# Autodesk Inventor assembly: 72 to 12 Single Stage Gearbox
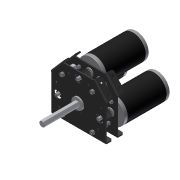
[picture p0: Inventor's stored thumbnail of the model, 180x180]
Saved by Autodesk Inventor 2013 (Build 170138000, 138)
## iProperties
Created: 2013-01-07
Part Number: 72 to 12 Single Stage Gearbox
Document SubType Name: Assembly
Designer: Nemo
Author: Nemo
## Documents named in this file (10)
- H:\Nemo\Documents\Robotics\VexPro\Gearbox - Single Reduction\72 to 12 Single Stage Gearbox.iam
- H:\Nemo\Documents\Robotics\VexPro\Gearbox - Single Reduction\72 single stage gearbox plate.ipt
- H:\Nemo\Documents\Robotics\VexPro\Fasteners\Hex Standoff 14-20 x1000.ipt
- H:\Nemo\Documents\Robotics\COTS Parts\Fasteners\14-20 SHCS x500.ipt
- H:\Nemo\Documents\Robotics\VexPro\Gearbox - Single Reduction\Single stage gearbox output shaft.ipt
- H:\Nemo\Documents\Robotics\VexPro\Bearings\Flanged Bearing - 0.5in Hex ID x 1.125in OD.ipt
- H:\Nemo\Documents\Robotics\VexPro\Bearings\Flanged Bearing - 0.5in Round ID x 1.125in OD.ipt
- H:\Nemo\Documents\Robotics\VexPro\Gears\Gear 20dp 500hex 72T Vex.ipt
- H:\Nemo\Documents\Robotics\VexPro\Gearbox - Single Reduction\500 Hex Coupler.ipt
- H:\Nemo\Documents\Robotics\VexPro\Gearbox - Single Reduction\CIM for Single Stage Vex Box.iam
## Components (22 placed, 9 different names)
1. 72 single stage gearbox plate:1 — Mate:1, Mate:2, Insert:1, Insert:2, Insert:3, Insert:4, Mate:3, Insert:9, Insert:10, Insert:11, Insert:12, Insert:13, Insert:18, Mate:4, Insert:19, Mate:5, Insert:20, Mate:6
2. 72 single stage gearbox plate:2 — Mate:1, Mate:2, Mate:3, Insert:5, Insert:6, Insert:7, Insert:8, Insert:14
3. Hex Standoff 14-20 x1000:1 — Insert:1
4. Hex Standoff 14-20 x1000:2 — Insert:4
5. Hex Standoff 14-20 x1000:3 — Insert:3
6. Hex Standoff 14-20 x1000:4 — Insert:2
7. 14-20 SHCS x500:1 — Insert:5
8. 14-20 SHCS x500:2 — Insert:6
9. 14-20 SHCS x500:3 — Insert:7
10. 14-20 SHCS x500:4 — Insert:8
11. 14-20 SHCS x500:5 — Insert:9
12. 14-20 SHCS x500:6 — Insert:12
13. 14-20 SHCS x500:7 — Insert:11
14. 14-20 SHCS x500:8 — Insert:10
15. Single stage gearbox output shaft:1 — Insert:15, Angle:1, Angle:2, Angle:3
16. Flanged Bearing - 0.5in Hex ID x 1.125in OD:1 — Insert:14, Angle:1, Insert:16
17. Flanged Bearing - 0.5in Round ID x 1.125in OD:1 — Insert:13, Insert:15
18. Gear 20dp 500hex 72T Vex:1 — Insert:16, Angle:2, Insert:17
19. 500 Hex Coupler:1 — Angle:3, Insert:17
20. CIM for Single Stage Vex Box:1 [sub-assembly] — Insert:18, Mate:4
21. CIM for Single Stage Vex Box:2 [sub-assembly] — Insert:19, Mate:5
22. CIM for Single Stage Vex Box:3 [sub-assembly] — Insert:20, Mate:6
## Relationships (29: Insert 20, Mate 6, Angle 3)
- Mate:1: 72 single stage gearbox plate:1 ↔ 72 single stage gearbox plate:2
- Mate:2: 72 single stage gearbox plate:1 ↔ 72 single stage gearbox plate:2
- Insert:1: 72 single stage gearbox plate:1 ↔ Hex Standoff 14-20 x1000:1
- Insert:2: 72 single stage gearbox plate:1 ↔ Hex Standoff 14-20 x1000:4
- Insert:3: 72 single stage gearbox plate:1 ↔ Hex Standoff 14-20 x1000:3
- Insert:4: 72 single stage gearbox plate:1 ↔ Hex Standoff 14-20 x1000:2
- Mate:3 (25.4 mm): 72 single stage gearbox plate:1 ↔ 72 single stage gearbox plate:2
- Insert:5: 72 single stage gearbox plate:2 ↔ 14-20 SHCS x500:1
- Insert:6: 72 single stage gearbox plate:2 ↔ 14-20 SHCS x500:2
- Insert:7: 72 single stage gearbox plate:2 ↔ 14-20 SHCS x500:3
- Insert:8: 72 single stage gearbox plate:2 ↔ 14-20 SHCS x500:4
- Insert:9: 72 single stage gearbox plate:1 ↔ 14-20 SHCS x500:5
- Insert:10: 72 single stage gearbox plate:1 ↔ 14-20 SHCS x500:8
- Insert:11: 72 single stage gearbox plate:1 ↔ 14-20 SHCS x500:7
- Insert:12: 72 single stage gearbox plate:1 ↔ 14-20 SHCS x500:6
- Insert:13: 72 single stage gearbox plate:1 ↔ Flanged Bearing - 0.5in Round ID x 1.125in OD:1
- Insert:14: 72 single stage gearbox plate:2 ↔ Flanged Bearing - 0.5in Hex ID x 1.125in OD:1
- Insert:15: Single stage gearbox output shaft:1 ↔ Flanged Bearing - 0.5in Round ID x 1.125in OD:1
- Angle:1 (0 deg): Single stage gearbox output shaft:1 ↔ Flanged Bearing - 0.5in Hex ID x 1.125in OD:1
- Insert:16: Flanged Bearing - 0.5in Hex ID x 1.125in OD:1 ↔ Gear 20dp 500hex 72T Vex:1
- Angle:2 (0 deg): Single stage gearbox output shaft:1 ↔ Gear 20dp 500hex 72T Vex:1
- Angle:3 (0 deg): Single stage gearbox output shaft:1 ↔ 500 Hex Coupler:1
- Insert:17: Gear 20dp 500hex 72T Vex:1 ↔ 500 Hex Coupler:1
- Insert:18: 72 single stage gearbox plate:1 ↔ CIM for Single Stage Vex Box:1
- Mate:4: 72 single stage gearbox plate:1 ↔ CIM for Single Stage Vex Box:1
- Insert:19: 72 single stage gearbox plate:1 ↔ CIM for Single Stage Vex Box:2
- Mate:5: 72 single stage gearbox plate:1 ↔ CIM for Single Stage Vex Box:2
- Insert:20: 72 single stage gearbox plate:1 ↔ CIM for Single Stage Vex Box:3
- Mate:6: 72 single stage gearbox plate:1 ↔ CIM for Single Stage Vex Box:3
